# Autodesk Inventor assembly: 42146-14
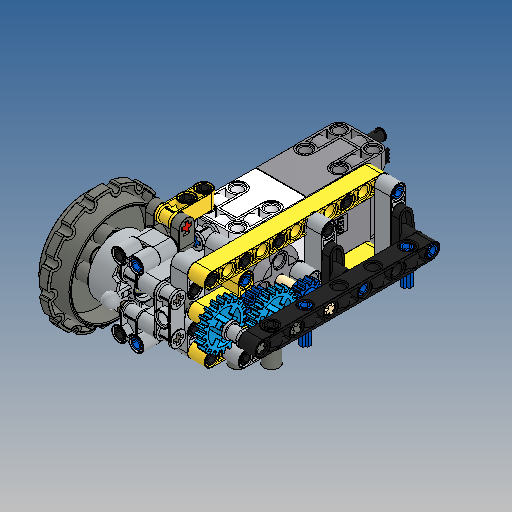
[picture p0: Inventor's stored thumbnail of the model, 512x512]
Saved by Autodesk Inventor 2025 (Build 290162010, 162A)
## iProperties
Created: 2024-11-18
Part Number: 42146-14
Material: Generisch
Document SubType Name: Assembly
Designer: hp.muther
Author: hp.muther
## Documents named in this file (33)
- D:\Inventor\Projekte\Muther\LEGO Technic\LEGO Technik - Raupenkran LR 13000 (42146)\42146-01-14.iam
- D:\Inventor\Projekte\Muther\LEGO Technic\LEGO Pieces\69730 - MOTOR, NR. 15.ipt
- D:\Inventor\Projekte\Muther\LEGO Technic\LEGO Pieces\43490-RadNabe.iam
- D:\Inventor\Projekte\Muther\LEGO Technic\LEGO Pieces\Pin's\18651-Black.ipt
- D:\Inventor\Projekte\Muther\LEGO Technic\LEGO Pieces\Pin's\6558-Blue.ipt
- D:\Inventor\Projekte\Muther\LEGO Technic\LEGO Pieces\Verbindungselemente\41678-DkBluishGray.ipt
- D:\Inventor\Projekte\Muther\LEGO Technic\LEGO Pieces\Achsen\32209-DkBluishGray.ipt
- D:\Inventor\Projekte\Muther\LEGO Technic\LEGO Pieces\Achsen\6587-DkTan.ipt
- D:\Inventor\Projekte\Muther\LEGO Technic\LEGO Pieces\Pin's\2780-Black.ipt
- D:\Inventor\Projekte\Muther\LEGO Technic\LEGO Pieces\Verbindungselemente\32291-LtBluishGray.ipt
- D:\Inventor\Projekte\Muther\LEGO Technic\LEGO Pieces\Diverses\52731-LtBluishGray.ipt
- D:\Inventor\Projekte\Muther\LEGO Technic\LEGO Pieces\Lochbalken\43857-LtBluishGray.ipt
- D:\Inventor\Projekte\Muther\LEGO Technic\LEGO Pieces\Verbindungselemente\32184-LtBluishGray.ipt
- D:\Inventor\Projekte\Muther\LEGO Technic\LEGO Pieces\Pin's\11214-Red.ipt
- D:\Inventor\Projekte\Muther\LEGO Technic\LEGO Pieces\Pin's\43093-Blue.ipt
- D:\Inventor\Projekte\Muther\LEGO Technic\LEGO Pieces\Achsen\32062-Red.ipt
- D:\Inventor\Projekte\Muther\LEGO Technic\LEGO Pieces\Rund\18654-DkBluishGray.ipt
- D:\Inventor\Projekte\Muther\LEGO Technic\LEGO Pieces\Verbindungselemente\42003-Yellow.ipt
- D:\Inventor\Projekte\Muther\LEGO Technic\LEGO Pieces\Rahmen, T-Stücke\60484-Yellow.ipt
- D:\Inventor\Projekte\Muther\LEGO Technic\LEGO Pieces\Achsen\87083-DkBluishGray.ipt
- D:\Inventor\Projekte\Muther\LEGO Technic\LEGO Pieces\Lochbalken\32525-Yellow.ipt
- D:\Inventor\Projekte\Muther\LEGO Technic\LEGO Pieces\Winkel\32526-LtBluishGray.ipt
- D:\Inventor\Projekte\Muther\LEGO Technic\LEGO Pieces\Zahnrad\69778-Blue.ipt
- D:\Inventor\Projekte\Muther\LEGO Technic\LEGO Pieces\Zahnrad\69779-DkAzure.ipt
- D:\Inventor\Projekte\Muther\LEGO Technic\LEGO Pieces\Rund\3713-LtBluishGray.ipt
- D:\Inventor\Projekte\Muther\LEGO Technic\LEGO Pieces\Achsen\99008-Tan.ipt
- D:\Inventor\Projekte\Muther\LEGO Technic\LEGO Pieces\Lochbalken\32316-LtBluishGray.ipt
- D:\Inventor\Projekte\Muther\LEGO Technic\LEGO Pieces\Verbindungselemente\15461-Black.ipt
- D:\Inventor\Projekte\Muther\LEGO Technic\LEGO Pieces\Lochbalken\73507-Black.ipt
- D:\Inventor\Projekte\Muther\LEGO Technic\LEGO Pieces\Verbindungselemente\48989-LtBluishGray.ipt
- D:\Inventor\Projekte\Muther\LEGO Technic\LEGO Pieces\Lochbalken\40490-DkBluishGray.ipt
- D:\Inventor\Projekte\Muther\LEGO Technic\LEGO Pieces\Räder, Raupe\45229-DkBluishGray.ipt
- D:\Inventor\Projekte\Muther\LEGO Technic\LEGO Pieces\Winkel\32140-LtBluishGray.ipt
## Components (84 placed, 32 different names)
1. 69730 - MOTOR, NR. 15:1 — Einfügen:29, Fluchtend:2, Einfügen:32, Einfügen:38, Fluchtend:4, Einfügen:42, Einfügen:43, Einfügen:45, Einfügen:46, Einfügen:49, Einfügen:53, Einfügen:75, Passend:28, Einfügen:76, Einfügen:77
2. 43490-RadNabe:1 [sub-assembly] — Einfügen:1, Einfügen:2, Einfügen:3, Einfügen:4, Einfügen:5, Einfügen:6, Passend:3, Passend:4, Passend:5, Einfügen:10, Einfügen:11, Einfügen:80, Passend:30
3. 18651-Black:1 — Einfügen:3, Passend:1, Passend:7
4. 18651-Black:2 — Einfügen:4, Passend:2, Passend:6
5. 6558-Blue:1 — Einfügen:1
6. 6558-Blue:2 — Einfügen:2
7. 41678-DkBluishGray:1 — Einfügen:5, Passend:2, Einfügen:33, Fluchtend:3, Einfügen:34
8. 41678-DkBluishGray:2 — Einfügen:6, Passend:1, Einfügen:39
9. 32209-DkBluishGray:1 — Einfügen:7, Passend:3, Passend:18, Passend:22
10. 6587-DkTan:1 — Einfügen:8, Passend:10, Passend:11
11. 6558-Blue:3 — Einfügen:12
12. 6558-Blue:4 — Einfügen:13, Passend:9, Passend:13
13. 6558-Blue:5 — Einfügen:14
14. 2780-Black:1 — Einfügen:15, Passend:8
15. 32316-LtBluishGray:3 — Einfügen:12, Einfügen:13, Einfügen:14, Einfügen:15, Einfügen:16, Einfügen:17, Einfügen:41, Einfügen:44
16. 32140-LtBluishGray:1 — Einfügen:16, Passend:9, Passend:10, Einfügen:24
17. 32140-LtBluishGray:2 — Einfügen:17, Passend:8, Einfügen:18, Einfügen:23, Einfügen:25, Pos. Zahnrad
18. 32291-LtBluishGray:1 — Einfügen:8, Einfügen:10, Passend:7
19. 52731-LtBluishGray:1 — Einfügen:7, Passend:4, Passend:5
20. 2780-Black:2 — Einfügen:19
21. 2780-Black:3 — Einfügen:20
22. 43857-LtBluishGray:1 — Einfügen:19, Einfügen:20, Einfügen:24, Fluchtend:1, Einfügen:48
23. 32184-LtBluishGray:1 — Einfügen:25, Passend:11
24. 32184-LtBluishGray:2 — Einfügen:26, Einfügen:27, Einfügen:28, Einfügen:29, Fluchtend:2, Passend:12
25. 11214-Red:1 — Einfügen:26
26. 43093-Blue:1 — Einfügen:27
27. 2780-Black:4 — Einfügen:31, Passend:12
28. 2780-Black:5 — Einfügen:30
29. 32062-Red:1 — Einfügen:34
30. 18654-DkBluishGray:1 — Einfügen:28
31. 18654-DkBluishGray:2 — Einfügen:37
32. 42003-Yellow:1 — Einfügen:30, Einfügen:31, Einfügen:32, Einfügen:33, Fluchtend:3
33. 42003-Yellow:2 — Einfügen:35, Einfügen:36, Einfügen:37, Einfügen:38, Fluchtend:4
34. 2780-Black:6 — Einfügen:35
35. 2780-Black:7 — Einfügen:36
36. 32062-Red:2 — Einfügen:39
37. 60484-Yellow:1 — Einfügen:40, Einfügen:41, Passend:13, Passend:19, Passend:20
38. 87083-DkBluishGray:1 — Einfügen:40, Passend:17, Passend:21
39. 2780-Black:8 — Einfügen:44
40. 2780-Black:9 — Einfügen:45, Passend:15
41. 2780-Black:10 — Einfügen:46
42. 2780-Black:11 — Einfügen:49
43. 2780-Black:12 — Einfügen:43, Passend:14
44. 2780-Black:13 — Einfügen:42
45. 32525-Yellow:1 — Einfügen:47, Passend:14, Einfügen:65, Einfügen:66
46. 32526-LtBluishGray:1 — Einfügen:50, Einfügen:51, Einfügen:52
47. 2780-Black:14 — Einfügen:50
48. 2780-Black:15 — Einfügen:51, Passend:16
49. 69778-Blue:1 — Passend:17, Passend:20, Passend:21, Drehung:1, Einfügen:56
50. 69779-DkAzure:1 — Passend:18, Passend:19, Passend:22, Drehung:1, Einfügen:55
51. 69779-DkAzure:2 — Einfügen:56, Drehung:2
52. 69778-Blue:2 — Einfügen:54, Drehung:2
53. 3713-LtBluishGray:1 — Einfügen:55
54. 99008-Tan:1 — Einfügen:53, Einfügen:54
55. 32525-Yellow:2 — Einfügen:48, Passend:15, Einfügen:52, Passend:16, Passend:25, Passend:26
56. 32316-LtBluishGray:1 — Einfügen:57, Einfügen:58, Einfügen:60, Passend:23, Einfügen:66
57. 32316-LtBluishGray:2 — Einfügen:62, Einfügen:63, Einfügen:64, Passend:24, Einfügen:65
58. 2780-Black:16 — Einfügen:57, Passend:25
59. 2780-Black:17 — Einfügen:58
60. 6558-Blue:6 — Einfügen:59, Passend:27
61. 6558-Blue:7 — Einfügen:61
62. 6558-Blue:8 — Einfügen:63
63. 6558-Blue:9 — Einfügen:62, Passend:26
64. 15461-Black:1 — Einfügen:59, Einfügen:60, Passend:23
65. 15461-Black:2 — Einfügen:61, Einfügen:64, Passend:24, Einfügen:71
66. 73507-Black:1 — Einfügen:67, Einfügen:68, Einfügen:69, Einfügen:70, Einfügen:71, Passend:27
67. 43093-Blue:2 — Einfügen:67
68. 43093-Blue:3 — Einfügen:68
69. 18654-DkBluishGray:3 — Einfügen:70
70. 2780-Black:18 — Einfügen:69
71. 2780-Black:19 — Einfügen:72
72. 2780-Black:20 — Einfügen:73
73. 18654-DkBluishGray:4 — Einfügen:74
74. 48989-LtBluishGray:1 — Einfügen:72, Einfügen:73, Einfügen:74, Einfügen:75, Passend:28, Einfügen:79
75. 6558-Blue:10 — Einfügen:77, Einfügen:78, Passend:29
76. 18654-DkBluishGray:5 — Einfügen:78
77. 18651-Black:3 — Einfügen:76
78. 40490-DkBluishGray:1 — Einfügen:79, Passend:29
79. 45229-DkBluishGray:1 — Einfügen:80, Passend:30, Pos. Zahnrad
80. 6587-DkTan:2
81. 32291-LtBluishGray:2 — Einfügen:11, Passend:6, Einfügen:18
82. 2780-Black:21 — Einfügen:21
83. 2780-Black:22 — Einfügen:22
84. 43857-LtBluishGray:2 — Einfügen:21, Einfügen:22, Einfügen:23, Fluchtend:1, Einfügen:47
## Relationships (117: Insert 80, Mate 31, Flush 4, RelateRotation 2)
- Pos. Zahnrad [Mate] (6.188 mm): 32140-LtBluishGray:2 ↔ 45229-DkBluishGray:1
- Einfügen:1 [Insert]: 43490-RadNabe:1 ↔ 6558-Blue:1
- Einfügen:2 [Insert]: 43490-RadNabe:1 ↔ 6558-Blue:2
- Einfügen:3 [Insert]: 43490-RadNabe:1 ↔ 18651-Black:1
- Einfügen:4 [Insert]: 43490-RadNabe:1 ↔ 18651-Black:2
- Einfügen:5 [Insert]: 43490-RadNabe:1 ↔ 41678-DkBluishGray:1
- Einfügen:6 [Insert]: 43490-RadNabe:1 ↔ 41678-DkBluishGray:2
- Passend:1 [Mate]: 18651-Black:1 ↔ 41678-DkBluishGray:2
- Passend:2 [Mate]: 18651-Black:2 ↔ 41678-DkBluishGray:1
- Einfügen:7 [Insert]: 32209-DkBluishGray:1 ↔ 52731-LtBluishGray:1
- Passend:3 [Mate]: 43490-RadNabe:1 ↔ 32209-DkBluishGray:1
- Passend:4 [Mate]: 43490-RadNabe:1 ↔ 52731-LtBluishGray:1
- Passend:5 [Mate]: 43490-RadNabe:1 ↔ 52731-LtBluishGray:1
- Einfügen:8 [Insert]: 6587-DkTan:1 ↔ 32291-LtBluishGray:1
- [Insert]: 6587-DkTan:2 ↔ 32291-LtBluishGray:2
- Einfügen:10 [Insert]: 43490-RadNabe:1 ↔ 32291-LtBluishGray:1
- Einfügen:11 [Insert]: 43490-RadNabe:1 ↔ 32291-LtBluishGray:2
- Passend:6 [Mate]: 18651-Black:2 ↔ 32291-LtBluishGray:2
- Passend:7 [Mate]: 18651-Black:1 ↔ 32291-LtBluishGray:1
- Einfügen:12 [Insert]: 6558-Blue:3 ↔ 32316-LtBluishGray:3
- Einfügen:13 [Insert]: 6558-Blue:4 ↔ 32316-LtBluishGray:3
- Einfügen:14 [Insert]: 6558-Blue:5 ↔ 32316-LtBluishGray:3
- Einfügen:15 [Insert]: 2780-Black:1 ↔ 32316-LtBluishGray:3
- Einfügen:16 [Insert]: 32316-LtBluishGray:3 ↔ 32140-LtBluishGray:1
- Einfügen:17 [Insert]: 32316-LtBluishGray:3 ↔ 32140-LtBluishGray:2
- Passend:8 [Mate]: 2780-Black:1 ↔ 32140-LtBluishGray:2
- Passend:9 [Mate]: 6558-Blue:4 ↔ 32140-LtBluishGray:1
- Einfügen:18 [Insert]: 32140-LtBluishGray:2 ↔ 32291-LtBluishGray:2
- Passend:10 [Mate]: 6587-DkTan:1 ↔ 32140-LtBluishGray:1
- Einfügen:19 [Insert]: 2780-Black:2 ↔ 43857-LtBluishGray:1
- Einfügen:20 [Insert]: 2780-Black:3 ↔ 43857-LtBluishGray:1
- Einfügen:21 [Insert]: 2780-Black:21 ↔ 43857-LtBluishGray:2
- Einfügen:22 [Insert]: 2780-Black:22 ↔ 43857-LtBluishGray:2
- Einfügen:23 [Insert]: 32140-LtBluishGray:2 ↔ 43857-LtBluishGray:2
- Einfügen:24 [Insert]: 32140-LtBluishGray:1 ↔ 43857-LtBluishGray:1
- Fluchtend:1 [Flush]: 43857-LtBluishGray:1 ↔ 43857-LtBluishGray:2
- Einfügen:25 [Insert]: 32140-LtBluishGray:2 ↔ 32184-LtBluishGray:1
- Passend:11 [Mate]: 6587-DkTan:1 ↔ 32184-LtBluishGray:1
- Einfügen:26 [Insert]: 32184-LtBluishGray:2 ↔ 11214-Red:1
- Einfügen:27 [Insert]: 32184-LtBluishGray:2 ↔ 43093-Blue:1
- Einfügen:28 [Insert]: 32184-LtBluishGray:2 ↔ 18654-DkBluishGray:1
- Einfügen:29 [Insert]: 69730 - MOTOR, NR. 15:1 ↔ 32184-LtBluishGray:2
- Fluchtend:2 [Flush]: 69730 - MOTOR, NR. 15:1 ↔ 32184-LtBluishGray:2
- Einfügen:30 [Insert]: 2780-Black:5 ↔ 42003-Yellow:1
- Einfügen:31 [Insert]: 2780-Black:4 ↔ 42003-Yellow:1
- Einfügen:32 [Insert]: 69730 - MOTOR, NR. 15:1 ↔ 42003-Yellow:1
- Passend:12 [Mate]: 32184-LtBluishGray:2 ↔ 2780-Black:4
- Einfügen:33 [Insert]: 41678-DkBluishGray:1 ↔ 42003-Yellow:1
- Fluchtend:3 [Flush]: 41678-DkBluishGray:1 ↔ 42003-Yellow:1
- Einfügen:34 [Insert]: 41678-DkBluishGray:1 ↔ 32062-Red:1
- Einfügen:35 [Insert]: 42003-Yellow:2 ↔ 2780-Black:6
- Einfügen:36 [Insert]: 42003-Yellow:2 ↔ 2780-Black:7
- Einfügen:37 [Insert]: 18654-DkBluishGray:2 ↔ 42003-Yellow:2
- Einfügen:38 [Insert]: 69730 - MOTOR, NR. 15:1 ↔ 42003-Yellow:2
- Fluchtend:4 [Flush]: 69730 - MOTOR, NR. 15:1 ↔ 42003-Yellow:2
- Einfügen:39 [Insert]: 41678-DkBluishGray:2 ↔ 32062-Red:2
- Einfügen:40 [Insert]: 60484-Yellow:1 ↔ 87083-DkBluishGray:1
- Einfügen:41 [Insert]: 32316-LtBluishGray:3 ↔ 60484-Yellow:1
- Passend:13 [Mate]: 6558-Blue:4 ↔ 60484-Yellow:1
- Einfügen:42 [Insert]: 69730 - MOTOR, NR. 15:1 ↔ 2780-Black:13
- Einfügen:43 [Insert]: 69730 - MOTOR, NR. 15:1 ↔ 2780-Black:12
- Einfügen:44 [Insert]: 32316-LtBluishGray:3 ↔ 2780-Black:8
- Einfügen:45 [Insert]: 69730 - MOTOR, NR. 15:1 ↔ 2780-Black:9
- Einfügen:46 [Insert]: 69730 - MOTOR, NR. 15:1 ↔ 2780-Black:10
- Einfügen:47 [Insert]: 32525-Yellow:1 ↔ 43857-LtBluishGray:2
- Einfügen:48 [Insert]: 43857-LtBluishGray:1 ↔ 32525-Yellow:2
- Passend:14 [Mate]: 2780-Black:12 ↔ 32525-Yellow:1
- Passend:15 [Mate]: 2780-Black:9 ↔ 32525-Yellow:2
- Einfügen:49 [Insert]: 69730 - MOTOR, NR. 15:1 ↔ 2780-Black:11
- Einfügen:50 [Insert]: 32526-LtBluishGray:1 ↔ 2780-Black:14
- Einfügen:51 [Insert]: 32526-LtBluishGray:1 ↔ 2780-Black:15
- Einfügen:52 [Insert]: 32526-LtBluishGray:1 ↔ 32525-Yellow:2
- Passend:16 [Mate]: 2780-Black:15 ↔ 32525-Yellow:2
- Passend:17 [Mate]: 87083-DkBluishGray:1 ↔ 69778-Blue:1
- Passend:18 [Mate]: 32209-DkBluishGray:1 ↔ 69779-DkAzure:1
- Passend:19 [Mate]: 60484-Yellow:1 ↔ 69779-DkAzure:1
- Passend:20 [Mate]: 60484-Yellow:1 ↔ 69778-Blue:1
- Passend:21 [Mate]: 87083-DkBluishGray:1 ↔ 69778-Blue:1
- Passend:22 [Mate]: 32209-DkBluishGray:1 ↔ 69779-DkAzure:1
- Drehung:1 [RelateRotation] (0.6 ul): 69778-Blue:1 ↔ 69779-DkAzure:1
- Einfügen:53 [Insert]: 69730 - MOTOR, NR. 15:1 ↔ 99008-Tan:1
- Einfügen:54 [Insert]: 69778-Blue:2 ↔ 99008-Tan:1
- Einfügen:55 [Insert]: 69779-DkAzure:1 ↔ 3713-LtBluishGray:1
- Einfügen:56 [Insert]: 69778-Blue:1 ↔ 69779-DkAzure:2
- Drehung:2 [RelateRotation] (0.6 ul): 69779-DkAzure:2 ↔ 69778-Blue:2
- Einfügen:57 [Insert]: 32316-LtBluishGray:1 ↔ 2780-Black:16
- Einfügen:58 [Insert]: 32316-LtBluishGray:1 ↔ 2780-Black:17
- Einfügen:59 [Insert]: 6558-Blue:6 ↔ 15461-Black:1
- Einfügen:60 [Insert]: 32316-LtBluishGray:1 ↔ 15461-Black:1
- Passend:23 [Mate]: 32316-LtBluishGray:1 ↔ 15461-Black:1
- Einfügen:61 [Insert]: 6558-Blue:7 ↔ 15461-Black:2
- Einfügen:62 [Insert]: 32316-LtBluishGray:2 ↔ 6558-Blue:9
- Einfügen:63 [Insert]: 32316-LtBluishGray:2 ↔ 6558-Blue:8
- Einfügen:64 [Insert]: 32316-LtBluishGray:2 ↔ 15461-Black:2
- Passend:24 [Mate]: 32316-LtBluishGray:2 ↔ 15461-Black:2
- Einfügen:65 [Insert]: 32525-Yellow:1 ↔ 32316-LtBluishGray:2
- Einfügen:66 [Insert]: 32525-Yellow:1 ↔ 32316-LtBluishGray:1
- Passend:25 [Mate]: 32525-Yellow:2 ↔ 2780-Black:16
- Passend:26 [Mate]: 32525-Yellow:2 ↔ 6558-Blue:9
- Einfügen:67 [Insert]: 73507-Black:1 ↔ 43093-Blue:2
- Einfügen:68 [Insert]: 73507-Black:1 ↔ 43093-Blue:3
- Einfügen:69 [Insert]: 73507-Black:1 ↔ 2780-Black:18
- Einfügen:70 [Insert]: 73507-Black:1 ↔ 18654-DkBluishGray:3
- Einfügen:71 [Insert]: 15461-Black:2 ↔ 73507-Black:1
- Passend:27 [Mate]: 6558-Blue:6 ↔ 73507-Black:1
- Einfügen:72 [Insert]: 2780-Black:19 ↔ 48989-LtBluishGray:1
- Einfügen:73 [Insert]: 2780-Black:20 ↔ 48989-LtBluishGray:1
- Einfügen:74 [Insert]: 18654-DkBluishGray:4 ↔ 48989-LtBluishGray:1
- Einfügen:75 [Insert]: 69730 - MOTOR, NR. 15:1 ↔ 48989-LtBluishGray:1
- Passend:28 [Mate]: 69730 - MOTOR, NR. 15:1 ↔ 48989-LtBluishGray:1
- Einfügen:76 [Insert]: 69730 - MOTOR, NR. 15:1 ↔ 18651-Black:3
- Einfügen:77 [Insert]: 69730 - MOTOR, NR. 15:1 ↔ 6558-Blue:10
- Einfügen:78 [Insert]: 6558-Blue:10 ↔ 18654-DkBluishGray:5
- Einfügen:79 [Insert]: 48989-LtBluishGray:1 ↔ 40490-DkBluishGray:1
- Passend:29 [Mate]: 6558-Blue:10 ↔ 40490-DkBluishGray:1
- Einfügen:80 [Insert]: 43490-RadNabe:1 ↔ 45229-DkBluishGray:1
- Passend:30 [Mate]: 43490-RadNabe:1 ↔ 45229-DkBluishGray:1
## Named parameters: d13_d12 = 0 mm, d30_d28 = 0 mm, d31_d29 = 0 mm
